# Autodesk Inventor assembly: Assembly2タミヤダンパー　上
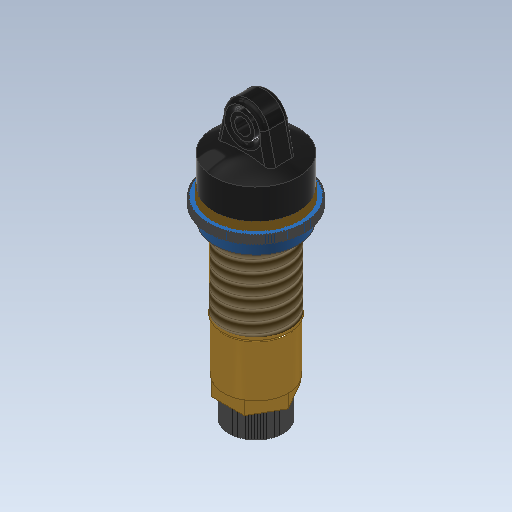
[picture p0: Inventor's stored thumbnail of the model, 512x512]
Saved by Autodesk Inventor 2020.2 (Build 242310000, 310)
## iProperties
Created: 2018-09-18
Part Number: Assembly2タミヤダンパー　上
Material: 一般
Document SubType Name: Assembly
Designer: 杉本　賢二郎
Author: 杉本　賢二郎
## Documents named in this file (7)
- C:\Users\aoyam\Desktop\SRDC_local\Inventor\二年機\Geminiβ\汎用部品\ダンパー\Assembly2タミヤダンパー　上.iam
- C:\Users\aoyam\Desktop\SRDC_local\Inventor\二年機\Geminiβ\汎用部品\ダンパー\タミヤダンパー部品1.ipt
- C:\Users\aoyam\Desktop\SRDC_local\Inventor\二年機\Geminiβ\汎用部品\ダンパー\タミヤダンパー部品2.ipt
- C:\Users\aoyam\Desktop\SRDC_local\Inventor\二年機\Geminiβ\汎用部品\ダンパー\タミヤダンパー部品3.ipt
- C:\Users\aoyam\Desktop\SRDC_local\Inventor\二年機\Geminiβ\汎用部品\ダンパー\タミヤダンパー部品4.ipt
- C:\Users\aoyam\Desktop\SRDC_local\Inventor\二年機\Geminiβ\汎用部品\ダンパー\タミヤダンパー部品8.ipt
- C:\Users\aoyam\Desktop\SRDC_local\Inventor\二年機\Geminiβ\汎用部品\ダンパー\タミヤダンパー部品6.ipt
## Components (6 placed, 6 different names)
1. タミヤダンパー部品1:1 — 挿入:1, 挿入:4
2. タミヤダンパー部品2:1 — 挿入:1, 挿入:2, メイト:1
3. タミヤダンパー部品3:1 — 挿入:2, 挿入:3
4. タミヤダンパー部品4:1 — メイト:1
5. タミヤダンパー部品8:1 — 挿入:4
6. タミヤダンパー部品6:1 — 挿入:3
## Relationships (5: Insert 4, Mate 1)
- 挿入:1 [Insert]: タミヤダンパー部品1:1 ↔ タミヤダンパー部品2:1
- 挿入:2 [Insert]: タミヤダンパー部品2:1 ↔ タミヤダンパー部品3:1
- 挿入:3 [Insert]: タミヤダンパー部品3:1 ↔ タミヤダンパー部品6:1
- メイト:1 [Mate]: タミヤダンパー部品2:1 ↔ タミヤダンパー部品4:1
- 挿入:4 [Insert]: タミヤダンパー部品1:1 ↔ タミヤダンパー部品8:1
